# Autodesk Inventor assembly: DesigningTop
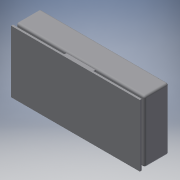
[picture p0: Inventor's stored thumbnail of the model, 180x180]
Saved by Autodesk Inventor 2017 (Build 210142000, 142)
## iProperties
Created: 2016-12-08
Part Number: DesigningTop
Document SubType Name: Assembly
Designer: SDL
Author: SDL
## Documents named in this file (4)
- C:\Users\SDL\Desktop\Current-Meter-Pcb-Fall-16-master\CAD\DesigningTop.iam
- C:\Users\SDL\Desktop\Current-Meter-Pcb-Fall-16-master\CAD\case3.ipt
- C:\Users\SDL\Desktop\Current-Meter-Pcb-Fall-16-master\CAD\top2.ipt
- C:\Users\SDL\Desktop\Current-Meter-Pcb-Fall-16-master\CAD\top2b.ipt
## Components (3 placed, 3 different names)
1. case3:1 — Flush:1
2. top2:1 — Flush:1, Rigid:1, Mate:1, Mate:2, Mate:3
3. top2b:1 — Rigid:1, Mate:1, Mate:2, Mate:3
## Relationships (5: Mate 3, Flush 1, WeldJoint 1)
- Flush:1: case3:1 ↔ top2:1
- Rigid:1 [WeldJoint]: top2:1 ↔ top2b:1
- Mate:1: top2:1 ↔ top2b:1
- Mate:2: top2:1 ↔ top2b:1
- Mate:3: top2:1 ↔ top2b:1
